# Autodesk Inventor assembly: Assembly shield 1_CPY2
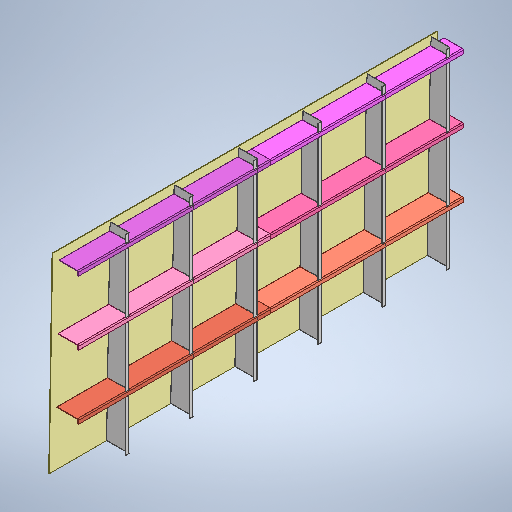
[picture p0: Inventor's stored thumbnail of the model, 512x512]
Saved by Autodesk Inventor 2026.2 (Build 302298000, 298)
## iProperties
Created: 2026-05-07
Part Number: Assembly shield 1_CPY2
Document SubType Name: Assembly
Designer: admin
Author: admin
## Documents named in this file (6)
- C:\Users\admin\Documents\Inventor\GBK-Gubkinskiy\Assembly shield 1_CPY2.iam
- C:\Users\admin\Documents\Inventor\GBK-Gubkinskiy\Part111_CPY2.ipt
- C:\Users\admin\Documents\Inventor\GBK-Gubkinskiy\stringer 1_CPY2.ipt
- C:\Users\admin\Documents\Inventor\GBK-Gubkinskiy\stringer 1.2_CPY2.ipt
- C:\Users\admin\Documents\Inventor\GBK-Gubkinskiy\Part2_CPY2.ipt
- C:\Users\admin\Documents\Inventor\GBK-Gubkinskiy\stringer 1.3_CPY2.ipt
## Components (13 placed, 5 different names)
1. Part111_CPY2:1 — Mate:1
2. stringer 1_CPY2:1 — Rigid:3, Rigid:1
3. stringer 1.2_CPY2:1 — Rigid:2, Rigid:5
4. stringer 1_CPY2:2 — Rigid:3
5. stringer 1.3_CPY2:1 — Rigid:4, Rigid:6
6. stringer 1.2_CPY2:2 — Rigid:5
7. stringer 1.3_CPY2:2 — Rigid:6
8. Part2_CPY2:1 — Mate:1, Rigid:2, Rigid:1, Rigid:4
9. Part2_CPY2:2
10. Part2_CPY2:3
11. Part2_CPY2:4
12. Part2_CPY2:5
13. Part2_CPY2:6
## Component patterns: (6 elements, first: Part2_CPY2:1)
## Relationships (7: WeldJoint 6, Mate 1)
- Mate:1: Part111_CPY2:1 ↔ Part2_CPY2:1
- Rigid:3 [WeldJoint]: stringer 1_CPY2:1 ↔ stringer 1_CPY2:2
- Rigid:2 [WeldJoint] (2 mm): stringer 1.2_CPY2:1 ↔ Part2_CPY2:1
- Rigid:1 [WeldJoint] (2 mm): stringer 1_CPY2:1 ↔ Part2_CPY2:1
- Rigid:4 [WeldJoint] (2 mm): stringer 1.3_CPY2:1 ↔ Part2_CPY2:1
- Rigid:5 [WeldJoint]: stringer 1.2_CPY2:1 ↔ stringer 1.2_CPY2:2
- Rigid:6 [WeldJoint]: stringer 1.3_CPY2:1 ↔ stringer 1.3_CPY2:2
